# Autodesk Inventor assembly: Expansor
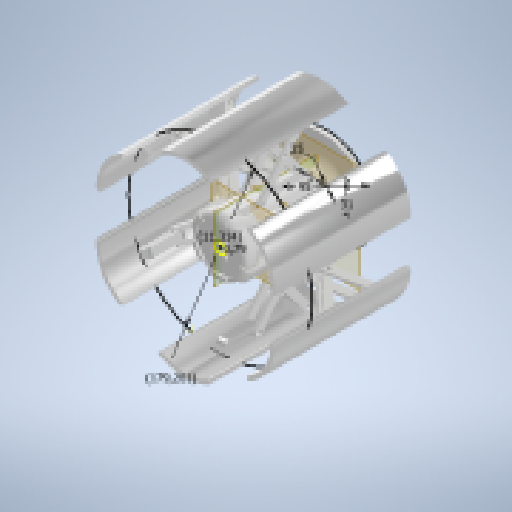
[picture p0: Inventor's stored thumbnail of the model, 512x512]
Saved by Autodesk Inventor 2024.3 (Build 283343000, 343)
## iProperties
RuleStatus: InUse
Created: 2024-11-12
Part Number: Expansor
Document SubType Name: Assembly
Designer: j.santaa
Author: j.santaa
## Documents named in this file (9)
- C:\Users\Usuario\OneDrive - Universidad de los andes\Robocol\Flotador\V2\Expansor\Expansor.iam
- C:\Users\Usuario\OneDrive - Universidad de los andes\Robocol\Flotador\V2\Expansor\Soporte.ipt
- C:\Users\Usuario\OneDrive - Universidad de los andes\Robocol\Flotador\V2\Expansor\Corredera I.ipt
- C:\Users\Usuario\OneDrive - Universidad de los andes\Robocol\Flotador\V2\Expansor\Corredor.ipt
- C:\Users\Usuario\OneDrive - Universidad de los andes\Robocol\Flotador\V2\Expansor\Paletas.ipt
- C:\Users\Usuario\OneDrive - Universidad de los andes\Robocol\Flotador\V2\Expansor\Corredera II.ipt
- C:\Users\Usuario\OneDrive - Universidad de los andes\Robocol\Flotador\Downloads\screw nut 8mm\screw nut 8mm.ipt
- C:\Users\Usuario\OneDrive - Universidad de los andes\Robocol\Flotador\V2\Expansor\Clavija.ipt
- C:\Users\Usuario\OneDrive - Universidad de los andes\Robocol\Flotador\V2\Expansor\Pieza.ipt
## Components (24 placed, 8 different names)
1. Soporte:1 — Ángulo:1, Coincidencia:2, De rotación:1, Cilíndrica:1, Coincidencia:3, Coincidencia:6
2. Corredor:1 — Cilíndrica:1, Coincidencia:3, De rotación:2, Rígido:1
3. screw nut 8mm:1 — Rígido:1
4. Clavija:1 — De rotación:3, Rígido:2, Rígido:3
5. Pieza:1 — Rígido:2
6. Pieza:2 — Rígido:3
7. Paletas:1 — Ángulo:1, Coincidencia:2, Coincidencia:5, Tangente:1, Coincidencia:6
8. Corredera II:1 — De rotación:1, Coincidencia:4, Tangente:1, De rotación:3
9. Corredera I:1 — De rotación:2, Coincidencia:4, Coincidencia:5
10. Paletas:2
11. Corredera II:2
12. Corredera I:2
13. Paletas:3
14. Corredera II:3
15. Corredera I:3
16. Paletas:4
17. Corredera II:4
18. Corredera I:4
19. Paletas:5
20. Corredera II:5
21. Corredera I:5
22. Paletas:6
23. Corredera II:6
24. Corredera I:6
## Component patterns: (6 elements, first: Paletas:1 + Corredera II:1 + Corredera I:1)
## Relationships (14: Mate 5, RevoluteJoint 3, WeldJoint 3, Angle 1, CylindricalJoint 1, Tangent 1)
- Ángulo:1 [Angle] (0 deg): Soporte:1 ↔ Paletas:1
- Coincidencia:2 [Mate]: Soporte:1 ↔ Paletas:1
- De rotación:1 [RevoluteJoint]: Soporte:1 ↔ Corredera II:1
- Cilíndrica:1 [CylindricalJoint]: Soporte:1 ↔ Corredor:1
- Coincidencia:3 [Mate]: Soporte:1 ↔ Corredor:1
- De rotación:2 [RevoluteJoint]: Corredor:1 ↔ Corredera I:1
- Coincidencia:4 [Mate]: Corredera II:1 ↔ Corredera I:1
- Coincidencia:5 [Mate]: Paletas:1 ↔ Corredera I:1
- Tangente:1: Paletas:1 ↔ Corredera II:1
- Rígido:1 [WeldJoint]: Corredor:1 ↔ screw nut 8mm:1
- De rotación:3 [RevoluteJoint] (0.05 mm): Clavija:1 ↔ Corredera II:1
- Rígido:2 [WeldJoint]: Clavija:1 ↔ Pieza:1
- Rígido:3 [WeldJoint]: Clavija:1 ↔ Pieza:2
- Coincidencia:6 [Mate] (0.235 mm): Soporte:1 ↔ Paletas:1
## Named parameters: LCorredera = 81 mm
